# Autodesk Inventor assembly: Rancidness
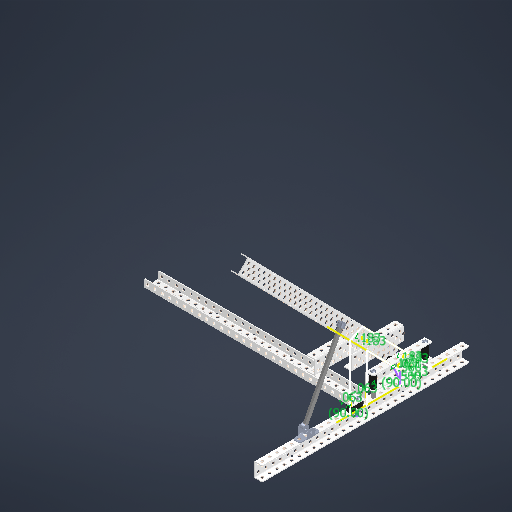
[picture p0: Inventor's stored thumbnail of the model, 512x512]
Saved by Autodesk Inventor 2025 (Build 290162000, 162)
## iProperties
Created: 2024-12-19
Part Number: Rancidness
Document SubType Name: Assembly
Designer: Juan
Author: Juan
## Documents named in this file (26)
- C:\Users\Juan\Documents\GitHub\ATUM-VRC-High-Stakes-CAD\Robot\Subassemblies\Rancidness.iam
- C:\Users\Juan\Documents\GitHub\ATUM-VRC-High-Stakes-CAD\VEX-CAD-Inventor\Structure\C Channel\Aluminum 1x2x1\Alu C 1x2x1x28.ipt
- C:\Users\Juan\Documents\GitHub\ATUM-VRC-High-Stakes-CAD\VEX-CAD-Inventor\Motion\Spacers\Spacer Nylon .500 OD\NSpacer Black .500 OD x .375.ipt
- C:\Users\Juan\Documents\GitHub\ATUM-VRC-High-Stakes-CAD\VEX-CAD-Inventor\Motion\Spacers\Spacer Nylon .500 OD.ipt
- C:\Users\Juan\Documents\GitHub\ATUM-VRC-High-Stakes-CAD\VEX-CAD-Inventor\Structure\C Channel\Aluminum 1x2x1\Alu C 1x2x1x8.ipt
- C:\Users\Juan\Documents\GitHub\ATUM-VRC-High-Stakes-CAD\VEX-CAD-Inventor\Structure\C Channel\Aluminum 1x2x1\Alu C 1x2x1x7.ipt
- C:\Users\Juan\Documents\GitHub\ATUM-VRC-High-Stakes-CAD\VEX-CAD-Inventor\Structure\Standoff\Standoff .50.ipt
- C:\Users\Juan\Documents\GitHub\ATUM-VRC-High-Stakes-CAD\VEX-CAD-Inventor\Structure\Standoff.ipt
- C:\Users\Juan\Documents\GitHub\ATUM-VRC-High-Stakes-CAD\VEX-CAD-Inventor\Motion\Spacers\Spacer Nylon .375 OD\NSpacer .375 OD x .500.ipt
- C:\Users\Juan\Documents\GitHub\ATUM-VRC-High-Stakes-CAD\VEX-CAD-Inventor\Motion\Spacers\Spacer Nylon .375 OD.ipt
- C:\Users\Juan\Documents\GitHub\ATUM-VRC-High-Stakes-CAD\VEX-CAD-Inventor\Motion\Spacers\Spacer Nylon .375 OD\NSpacer .375 OD x .375.ipt
- C:\Users\Juan\Documents\GitHub\ATUM-VRC-High-Stakes-CAD\VEX-CAD-Inventor\Structure\C Channel\Aluminum 1x2x1\Alu C 1x2x1x29.ipt
- C:\Users\Juan\Documents\GitHub\ATUM-VRC-High-Stakes-CAD\VEX-CAD-Inventor\Motion\Pneumatics\Legacy - SMC Pneumatics\Cylinder Rod Pivot.ipt
- C:\Users\Juan\Documents\GitHub\ATUM-VRC-High-Stakes-CAD\VEX-CAD-Inventor\Motion\Shaft LS\Shaft Collar Metal\Shaft Collar No Screw.ipt
- C:\Users\Juan\Documents\GitHub\ATUM-VRC-High-Stakes-CAD\VEX-CAD-Inventor\Structure\Standoff\Standoff 4.00.ipt
- C:\Users\Juan\Documents\GitHub\ATUM-VRC-High-Stakes-CAD\VEX-CAD-Inventor\Structure\Standoff\Standoff 1.00.ipt
- C:\Users\Juan\Documents\GitHub\ATUM-VRC-High-Stakes-CAD\VEX-CAD-Inventor\Structure\Hardware\Screw Steel - Star\SScrew Star Smooth .750.ipt
- C:\Users\Juan\Documents\GitHub\ATUM-VRC-High-Stakes-CAD\VEX-CAD-Inventor\Structure\Hardware\Screw Steel - Star.ipt
- C:\Users\Juan\Documents\GitHub\ATUM-VRC-High-Stakes-CAD\VEX-CAD-Inventor\Structure\Hardware\Nut Nylock.ipt
- C:\Users\Juan\Documents\GitHub\ATUM-VRC-High-Stakes-CAD\VEX-CAD-Inventor\Motion\Spacers\Washer Teflon\TWasher .375 OD x .03125.ipt
- C:\Users\Juan\Documents\GitHub\ATUM-VRC-High-Stakes-CAD\VEX-CAD-Inventor\Motion\Spacers\Washer Teflon.ipt
- C:\Users\Juan\Documents\GitHub\ATUM-VRC-High-Stakes-CAD\VEX-CAD-Inventor\Structure\Hardware\Nut Thin Nylock.ipt
- C:\Users\Juan\Documents\GitHub\ATUM-VRC-High-Stakes-CAD\VEX-CAD-Inventor\Structure\Hardware\Screw Steel - Star\SScrew Star Smooth .500.ipt
- C:\Users\Juan\Documents\GitHub\ATUM-VRC-High-Stakes-CAD\VEX-CAD-Inventor\Motion\Spacers\Spacer Nylon .375 OD\NSpacer .375 OD x .125.ipt
- C:\Users\Juan\Documents\GitHub\ATUM-VRC-High-Stakes-CAD\VEX-CAD-Inventor\Structure\Hardware\Screw Steel - Star\SScrew Star Smooth 1.250.ipt
- C:\Users\Juan\Documents\GitHub\ATUM-VRC-High-Stakes-CAD\VEX-CAD-Inventor\Structure\Hardware\Screw Steel - Star\SScrew Star Smooth .250.ipt
## Components (33 placed, 20 different names)
1. Alu C 1x2x1x28:1
2. Alu C 1x2x1x28:2
3. NSpacer Black .500 OD x .375:1
4. NSpacer Black .500 OD x .375:2
5. Alu C 1x2x1x8:1
6. Alu C 1x2x1x7:1
7. Alu C 1x2x1x7:2
8. Standoff .50:1
9. Standoff .50:2
10. NSpacer .375 OD x .500:1
11. NSpacer .375 OD x .375:2
12. NSpacer .375 OD x .500:3
13. NSpacer .375 OD x .375:4
14. Alu C 1x2x1x29:1
15. Cylinder Rod Pivot:1
16. Shaft Collar No Screw:1
17. Standoff 4.00:3
18. Standoff 1.00:4
19. Shaft Collar No Screw:2
20. SScrew Star Smooth .750:1
21. SScrew Star Smooth .750:2
22. Nut Nylock:1
23. Nut Nylock:2
24. Shaft Collar No Screw:3
25. TWasher .375 OD x .03125:1
26. Shaft Collar No Screw:4
27. Nut Thin Nylock:1
28. SScrew Star Smooth .500:3
29. NSpacer .375 OD x .125:5
30. SScrew Star Smooth 1.250:4
31. SScrew Star Smooth 1.250:5
32. SScrew Star Smooth .250:6
33. SScrew Star Smooth .250:7
## Relationships (50: Mate 38, WeldJoint 8, RevoluteJoint 4)
- [Mate]: Alu C 1x2x1x28:1 ↔ Alu C 1x2x1x28:2
- [Mate]: Alu C 1x2x1x28:1 ↔ Alu C 1x2x1x28:2
- [Mate]: Alu C 1x2x1x28:1 ↔ NSpacer Black .500 OD x .375:1
- [Mate]: Alu C 1x2x1x28:2 ↔ NSpacer Black .500 OD x .375:1
- [Mate]: Alu C 1x2x1x28:1 ↔ NSpacer Black .500 OD x .375:1
- [Mate]: Alu C 1x2x1x28:1 ↔ NSpacer Black .500 OD x .375:2
- [Mate]: Alu C 1x2x1x28:2 ↔ NSpacer Black .500 OD x .375:2
- [Mate]: Alu C 1x2x1x28:1 ↔ Alu C 1x2x1x8:1
- [Mate]: Alu C 1x2x1x28:1 ↔ Alu C 1x2x1x8:1
- [Mate] (12.7 mm): Alu C 1x2x1x28:1 ↔ Alu C 1x2x1x8:1
- [Mate]: Alu C 1x2x1x28:1 ↔ Standoff .50:1
- [Mate]: Alu C 1x2x1x28:1 ↔ Standoff .50:2
- [Mate]: Alu C 1x2x1x28:1 ↔ Standoff .50:2
- [Mate]: Alu C 1x2x1x28:1 ↔ Standoff .50:1
- [Mate]: NSpacer .375 OD x .500:1 ↔ NSpacer .375 OD x .375:2
- [Mate]: Alu C 1x2x1x8:1 ↔ NSpacer .375 OD x .500:1
- [Mate]: Alu C 1x2x1x8:1 ↔ NSpacer .375 OD x .500:1
- [Mate]: NSpacer .375 OD x .500:1 ↔ NSpacer .375 OD x .375:2
- [Mate]: NSpacer .375 OD x .500:3 ↔ NSpacer .375 OD x .375:4
- [Mate]: NSpacer .375 OD x .500:3 ↔ NSpacer .375 OD x .375:4
- [Mate]: Alu C 1x2x1x8:1 ↔ NSpacer .375 OD x .500:3
- [Mate]: Alu C 1x2x1x8:1 ↔ NSpacer .375 OD x .500:3
- [Mate]: Alu C 1x2x1x8:1 ↔ Alu C 1x2x1x29:1
- [Mate]: Alu C 1x2x1x28:1 ↔ Cylinder Rod Pivot:1
- [Mate]: Alu C 1x2x1x28:1 ↔ Cylinder Rod Pivot:1
- [Mate]: Alu C 1x2x1x28:1 ↔ Cylinder Rod Pivot:1
- [Mate]: Cylinder Rod Pivot:1 ↔ Shaft Collar No Screw:1
- [Mate]: Cylinder Rod Pivot:1 ↔ Shaft Collar No Screw:1
- [Mate]: Shaft Collar No Screw:1 ↔ Standoff 4.00:3
- [Mate]: Shaft Collar No Screw:1 ↔ Standoff 4.00:3
- [Mate]: Standoff 4.00:3 ↔ Standoff 1.00:4
- [Mate]: Standoff 4.00:3 ↔ Standoff 1.00:4
- [Mate]: Standoff 1.00:4 ↔ Shaft Collar No Screw:2
- [Mate]: Alu C 1x2x1x29:1 ↔ Shaft Collar No Screw:2
- [Mate] (1.5875 mm): Standoff 1.00:4 ↔ Shaft Collar No Screw:2
- [Mate]: Alu C 1x2x1x29:1 ↔ NSpacer .375 OD x .125:5
- [Mate]: Alu C 1x2x1x8:1 ↔ NSpacer .375 OD x .125:5
- [Mate]: Alu C 1x2x1x29:1 ↔ NSpacer .375 OD x .125:5
- [RevoluteJoint]: Alu C 1x2x1x28:2 ↔ SScrew Star Smooth .750:2
- [RevoluteJoint]: Alu C 1x2x1x28:2 ↔ SScrew Star Smooth .750:1
- [WeldJoint]: Alu C 1x2x1x28:1 ↔ Nut Nylock:2
- [RevoluteJoint]: Alu C 1x2x1x28:1 ↔ Nut Nylock:1
- [WeldJoint]: Alu C 1x2x1x8:1 ↔ TWasher .375 OD x .03125:1
- [WeldJoint]: Shaft Collar No Screw:3 ↔ TWasher .375 OD x .03125:1
- [WeldJoint]: Alu C 1x2x1x8:1 ↔ Nut Thin Nylock:1
- [RevoluteJoint]: Alu C 1x2x1x8:1 ↔ SScrew Star Smooth .500:3
- [WeldJoint]: Alu C 1x2x1x8:1 ↔ SScrew Star Smooth 1.250:5
- [WeldJoint]: Alu C 1x2x1x8:1 ↔ SScrew Star Smooth 1.250:4
- [WeldJoint]: Alu C 1x2x1x28:1 ↔ SScrew Star Smooth .250:7
- [WeldJoint]: Alu C 1x2x1x28:1 ↔ SScrew Star Smooth .250:6
## Named parameters: d1013_d1012 = 0 mm, d1014_d1009 = 0 mm
